# Autodesk Inventor assembly: Full Mars Robot
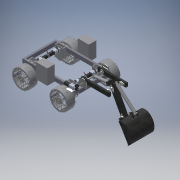
[picture p0: Inventor's stored thumbnail of the model, 180x180]
Saved by Autodesk Inventor 2019 (Build 230136000, 136)
## iProperties
Created: 2018-11-29
Part Number: Full Mars Robot
Document SubType Name: Assembly
Designer: Alex Barnett
Author: Alex Barnett
## Documents named in this file (3)
- C:\Users\Alex Barnett\Documents\Machine Design\PR2\CAD\Full Mars Robot.iam
- C:\Users\Alex Barnett\Documents\Machine Design\PR2\CAD\Frame\Frame Assembly.iam
- C:\Users\Alex Barnett\Documents\Machine Design\PR2\CAD\Backhoe.iam
## Components (2 placed, 2 different names)
1. Frame Assembly:1 [sub-assembly] — Mate:1, Mate:2, Flush:1
2. Backhoe:1 [sub-assembly] — Mate:1, Mate:2, Flush:1
## Relationships (3: Mate 2, Flush 1)
- Mate:1: Frame Assembly:1 ↔ Backhoe:1
- Mate:2: Frame Assembly:1 ↔ Backhoe:1
- Flush:1: Frame Assembly:1 ↔ Backhoe:1
